# Autodesk Inventor assembly: table
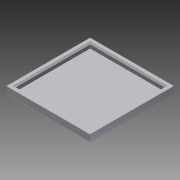
[picture p0: Inventor's stored thumbnail of the model, 180x180]
Saved by Autodesk Inventor 2013 (Build 170138000, 138)
## iProperties
Created: 2012-10-20
Part Number: table
Document SubType Name: Weldment
Designer: Istvan
Weld Material: Welded Aluminum-6061
Mass: 18318.1 g
Surface Area: 68009.8 cm^2
Volume: 8886.11 cm^3
Density: 2.06143 g/cm^3
Author: Istvan
## Documents named in this file (7)
- D:\GitHub\Crown-Fire\CAD\Frame\Table\table.iam
- D:\GitHub\Crown-Fire\CAD\Frame\Table\tableBottom.ipt
- D:\GitHub\Crown-Fire\CAD\Frame\Table\tableSide.ipt
- C:\Users\istvan.burbank\Documents\GitHub\Crown-Fire\CAD\Templates\squareTube1.5x2.ipt
- D:\GitHub\Crown-Fire\CAD\Frame\Table\slatHolder.ipt
- D:\GitHub\Crown-Fire\CAD\Frame\Table\slatHolderDiag.ipt
- D:\GitHub\Crown-Fire\CAD\Frame\Table\slatHolderShort.ipt
## Components (10 placed, 5 different names)
1. tableBottom:1 — Mate:9, Mate:10, Mate:11, Mate:14, Mate:15, Mate:20, Flush:5, Flush:7, Mate:23, Mate:24
2. tableSide:1 — Mate:5, Mate:6, Flush:1, Mate:7, Mate:8, Mate:9, Mate:21, Mate:28
3. tableSide:2 — Mate:4, Mate:6, Flush:1, Flush:2, Mate:8, Mate:10
4. tableSide:3 — Mate:2, Mate:5, Flush:3, Mate:7, Mate:22
5. tableSide:4 — Mate:2, Mate:4, Flush:2, Flush:3, Mate:11, Mate:27
6. slatHolder:2 — Mate:14, Flush:5, Mate:22
7. slatHolder:4 — Mate:15, Flush:7, Mate:21, Mate:25, Mate:26
8. slatHolderDiag:5 — Mate:20
9. slatHolderShort:6 — Mate:23, Mate:26, Mate:27
10. slatHolderShort:7 — Mate:24, Mate:25, Mate:28
## Relationships (25: Mate 20, Flush 5)
- Mate:2: tableSide:3 ↔ tableSide:4
- Mate:4: tableSide:2 ↔ tableSide:4
- Mate:5: tableSide:1 ↔ tableSide:3
- Mate:6: tableSide:1 ↔ tableSide:2
- Flush:1: tableSide:1 ↔ tableSide:2
- Flush:2: tableSide:2 ↔ tableSide:4
- Flush:3: tableSide:3 ↔ tableSide:4
- Mate:7: tableSide:1 ↔ tableSide:3
- Mate:8: tableSide:1 ↔ tableSide:2
- Mate:9: tableBottom:1 ↔ tableSide:1
- Mate:10: tableBottom:1 ↔ tableSide:2
- Mate:11: tableBottom:1 ↔ tableSide:4
- Mate:14: tableBottom:1 ↔ slatHolder:2
- Mate:15: tableBottom:1 ↔ slatHolder:4
- Mate:20: tableBottom:1 ↔ slatHolderDiag:5
- Flush:5: tableBottom:1 ↔ slatHolder:2
- Flush:7: tableBottom:1 ↔ slatHolder:4
- Mate:21: tableSide:1 ↔ slatHolder:4
- Mate:22: tableSide:3 ↔ slatHolder:2
- Mate:23: tableBottom:1 ↔ slatHolderShort:6
- Mate:24: tableBottom:1 ↔ slatHolderShort:7
- Mate:25: slatHolder:4 ↔ slatHolderShort:7
- Mate:26: slatHolder:4 ↔ slatHolderShort:6
- Mate:27: tableSide:4 ↔ slatHolderShort:6
- Mate:28: tableSide:1 ↔ slatHolderShort:7
